# Autodesk Inventor assembly: Console
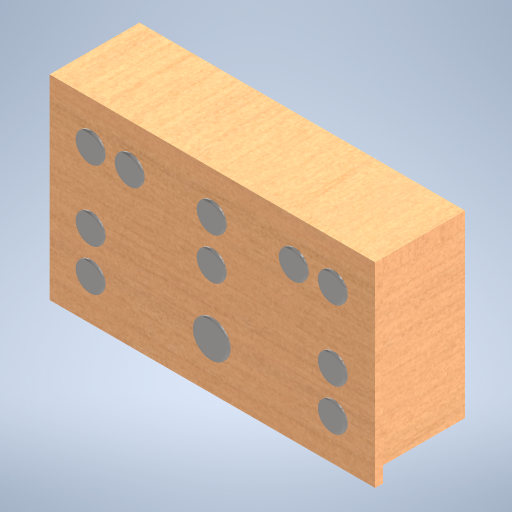
[picture p0: Inventor's stored thumbnail of the model, 512x512]
Saved by Autodesk Inventor 2024 (Build 280153000, 153)
## iProperties
Created: 2024-05-02
Part Number: Console
Document SubType Name: Assembly
Designer: haniv
Author: haniv
## Documents named in this file (8)
- C:\Users\haniv\Desktop\Unterlagen\Projekte\7_Segment_Anzeige\ScoreDisplay\CAD\Console.iam
- C:\Users\haniv\Desktop\Unterlagen\Projekte\7_Segment_Anzeige\ScoreDisplay\CAD\Components\Grundplatte_Konsole.ipt
- C:\Users\haniv\Desktop\Unterlagen\Projekte\7_Segment_Anzeige\ScoreDisplay\CAD\Components\Querseite_Konsole.ipt
- C:\Users\haniv\Desktop\Unterlagen\Projekte\7_Segment_Anzeige\ScoreDisplay\CAD\Components\Längsseite_Konsole.ipt
- C:\Users\haniv\Desktop\Unterlagen\Projekte\7_Segment_Anzeige\ScoreDisplay\CAD\Components\Oberseite_Konsole.ipt
- C:\Users\haniv\Desktop\Unterlagen\Projekte\7_Segment_Anzeige\ScoreDisplay\CAD\Components\Druckknopf_Konsole_groß.ipt
- C:\Users\haniv\Desktop\Unterlagen\Projekte\7_Segment_Anzeige\ScoreDisplay\CAD\Components\Druckknopf_Konsole_klein.ipt
- C:\Users\haniv\Desktop\Unterlagen\Projekte\7_Segment_Anzeige\ScoreDisplay\CAD\Components\Druckknopf_Konsole_klein_MIR.ipt
## Components (17 placed, 7 different names)
1. Grundplatte_Konsole:1 — Passend:1, Fluchtend:1, Fluchtend:2, Passend:2, Passend:3, Passend:4, Fluchtend:4
2. Querseite_Konsole:1 — Passend:4, Passend:5, Fluchtend:3, Fluchtend:5, Fluchtend:7
3. Querseite_Konsole:2 — Passend:3, Fluchtend:4, Passend:6, Passend:7, Passend:8
4. Längsseite_Konsole:1 — Passend:2, Passend:7, Fluchtend:5
5. Längsseite_Konsole:2 — Passend:1, Fluchtend:1, Fluchtend:2, Passend:5, Fluchtend:3, Passend:6, Fluchtend:6
6. Oberseite_Konsole:1 — Passend:8, Fluchtend:6, Fluchtend:7, Passend:9, Passend:10, Passend:11, Passend:12, Passend:13, Passend:14, Passend:16, Passend:17
7. Druckknopf_Konsole_groß:1 — Passend:9, Passend:10
8. Druckknopf_Konsole_klein_MIR:1
9. Druckknopf_Konsole_klein_MIR:2
10. Druckknopf_Konsole_klein_MIR:3
11. Druckknopf_Konsole_klein_MIR:4
12. Druckknopf_Konsole_klein:1 — Passend:11, Passend:12
13. Druckknopf_Konsole_klein:2
14. Druckknopf_Konsole_klein:3 — Passend:13, Passend:14
15. Druckknopf_Konsole_klein:4
16. Druckknopf_Konsole_klein:5 — Passend:16, Passend:17
17. Druckknopf_Konsole_klein:6
## Component patterns: (2 elements, first: Druckknopf_Konsole_klein:1), (2 elements, first: Druckknopf_Konsole_klein:3), (2 elements, first: Druckknopf_Konsole_klein:5)
## Relationships (23: Mate 16, Flush 7)
- Passend:1 [Mate]: Grundplatte_Konsole:1 ↔ Längsseite_Konsole:2
- Fluchtend:1 [Flush]: Grundplatte_Konsole:1 ↔ Längsseite_Konsole:2
- Fluchtend:2 [Flush]: Grundplatte_Konsole:1 ↔ Längsseite_Konsole:2
- Passend:2 [Mate]: Grundplatte_Konsole:1 ↔ Längsseite_Konsole:1
- Passend:3 [Mate]: Grundplatte_Konsole:1 ↔ Querseite_Konsole:2
- Passend:4 [Mate]: Grundplatte_Konsole:1 ↔ Querseite_Konsole:1
- Passend:5 [Mate]: Querseite_Konsole:1 ↔ Längsseite_Konsole:2
- Fluchtend:3 [Flush]: Querseite_Konsole:1 ↔ Längsseite_Konsole:2
- Fluchtend:4 [Flush]: Grundplatte_Konsole:1 ↔ Querseite_Konsole:2
- Passend:6 [Mate]: Querseite_Konsole:2 ↔ Längsseite_Konsole:2
- Passend:7 [Mate]: Querseite_Konsole:2 ↔ Längsseite_Konsole:1
- Fluchtend:5 [Flush]: Querseite_Konsole:1 ↔ Längsseite_Konsole:1
- Passend:8 [Mate]: Querseite_Konsole:2 ↔ Oberseite_Konsole:1
- Fluchtend:6 [Flush]: Längsseite_Konsole:2 ↔ Oberseite_Konsole:1
- Fluchtend:7 [Flush]: Querseite_Konsole:1 ↔ Oberseite_Konsole:1
- Passend:9 [Mate]: Oberseite_Konsole:1 ↔ Druckknopf_Konsole_groß:1
- Passend:10 [Mate]: Oberseite_Konsole:1 ↔ Druckknopf_Konsole_groß:1
- Passend:11 [Mate]: Oberseite_Konsole:1 ↔ Druckknopf_Konsole_klein:1
- Passend:12 [Mate]: Oberseite_Konsole:1 ↔ Druckknopf_Konsole_klein:1
- Passend:13 [Mate]: Oberseite_Konsole:1 ↔ Druckknopf_Konsole_klein:3
- Passend:14 [Mate]: Oberseite_Konsole:1 ↔ Druckknopf_Konsole_klein:3
- Passend:16 [Mate]: Oberseite_Konsole:1 ↔ Druckknopf_Konsole_klein:5
- Passend:17 [Mate]: Oberseite_Konsole:1 ↔ Druckknopf_Konsole_klein:5
